# Autodesk Inventor assembly: EDMPumpRegionAssembly
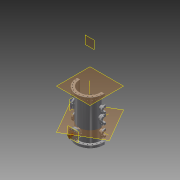
[picture p0: Inventor's stored thumbnail of the model, 180x180]
Saved by Autodesk Inventor 2015 (Build 190159000, 159)
## iProperties
Created: 2014-03-24
Part Number: EDMPumpRegionAssembly
Document SubType Name: Assembly
Designer: jad211
Author: jad211
## Documents named in this file (8)
- C:\CADFiles\EDM Machine\EDM New Pumping Region\EDMPumpRegionAssembly.iam
- C:\CADFiles\EDM Machine\EDM New Pumping Region\NewHorn.ipt
- C:\CADFiles\EDM Machine\EDM New Pumping Region\WG18FLANGECutDown.ipt
- C:\CADFiles\EDM Machine\EDM Middle Shield\EDM Middle shield.ipt
- C:\CADFiles\EDM Machine\EDM Inner Shield\Inner Shield.iam
- C:\CADFiles\EDM Machine\EDM Beamline\Chamber parts\hudson chamber actual size.ipt
- C:\CADFiles\EDM Machine\EDM New Pumping Region\FlangedWaveguide.iam
- C:\CADFiles\EDM Machine\EDM New Pumping Region\3-38sWithWG18Hole.ipt
## Components (7 placed, 7 different names)
1. EDM Middle shield:1 — Mate:8, Flush:11
2. Inner Shield:1 [sub-assembly] — Flush:14, Mate:10, Flush:13, Flush:19
3. hudson chamber actual size:1 — Mate:12, Flush:15, Angle:1, Mate:13, Mate:24
4. NewHorn:1 — Mate:14, Angle:2, Flush:17, Mate:17, Mate:18, Mate:19, Mate:21, Flush:20
5. WG18FLANGECutDown:1 — Flush:17, Mate:18, Mate:19, Mate:20
6. FlangedWaveguide:2 [sub-assembly] — Mate:17, Mate:20, Mate:21, Mate:22, Mate:23
7. 3-38sWithWG18Hole:1 — Mate:22, Mate:23, Mate:24
## Relationships (24: Mate 13, Flush 9, Angle 2)
- Flush:8 (3 mm)
- Mate:8: EDM Middle shield:1
- Flush:11 (158.75 mm): EDM Middle shield:1
- Flush:14 (64.29 mm): Inner Shield:1
- Mate:10: Inner Shield:1
- Flush:13: Inner Shield:1
- Mate:12: hudson chamber actual size:1
- Flush:15: hudson chamber actual size:1
- Flush:16 (-304.8 mm)
- Angle:1 (0 deg): hudson chamber actual size:1
- Mate:13: hudson chamber actual size:1
- Mate:14: NewHorn:1
- Angle:2 (0 deg): NewHorn:1
- Flush:17: NewHorn:1 ↔ WG18FLANGECutDown:1
- Mate:17: NewHorn:1 ↔ FlangedWaveguide:2
- Flush:19 (90 mm): Inner Shield:1
- Mate:18: NewHorn:1 ↔ WG18FLANGECutDown:1
- Mate:19: NewHorn:1 ↔ WG18FLANGECutDown:1
- Mate:20: WG18FLANGECutDown:1 ↔ FlangedWaveguide:2
- Mate:21: NewHorn:1 ↔ FlangedWaveguide:2
- Flush:20 (-5 mm): NewHorn:1
- Mate:22: FlangedWaveguide:2 ↔ 3-38sWithWG18Hole:1
- Mate:23: FlangedWaveguide:2 ↔ 3-38sWithWG18Hole:1
- Mate:24: hudson chamber actual size:1 ↔ 3-38sWithWG18Hole:1
